# Autodesk Inventor assembly: RC Car Final Model
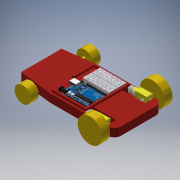
[picture p0: Inventor's stored thumbnail of the model, 180x180]
Saved by Autodesk Inventor 2019 (Build 230136000, 136)
## iProperties
Created: 2020-12-19
Part Number: RC Car Final Model
Document SubType Name: Assembly
Designer: wahid
Author: wahid
## Documents named in this file (9)
- C:\Users\wahid\Desktop\rc\Final Assembly\RC Car Final Model.iam
- C:\Users\wahid\Desktop\rc\Parts\Chassis\RC_Chassis.ipt
- C:\Users\wahid\Desktop\rc\Parts\Arduino\ardino.ipt
- C:\Users\wahid\Desktop\rc\Parts\Bread Board\Breadboard part\HalfBreadboard.ipt
- C:\Users\wahid\Desktop\rc\Parts\Motor\Original\Hobby_GearMotor.ipt
- C:\Users\wahid\Desktop\rc\Parts\Axle\Back Axle\Back Axle.ipt
- C:\Users\wahid\Desktop\rc\Parts\Wheel\Back Wheel\Back Wheel.ipt
- C:\Users\wahid\Desktop\rc\Parts\Axle\Front Axle\Front Axle.ipt
- C:\Users\wahid\Desktop\rc\Parts\Wheel\Front Wheel\Front Wheel.ipt
## Components (12 placed, 8 different names)
1. RC_Chassis:1 — Mate:3, Mate:4, Mate:5, Flush:1, Mate:6, Mate:7, Flush:2, Mate:8, Mate:12, Mate:13, Mate:14, Mate:15
2. HalfBreadboard:1 — Mate:3, Mate:4, Mate:12, Flush:4
3. Hobby_GearMotor:1 — Mate:5, Flush:1, Mate:6, Mate:9
4. Hobby_GearMotor:2 — Mate:7, Flush:2, Mate:8, Mate:10
5. Back Axle:1 — Mate:9, Insert:1
6. Back Axle:2 — Mate:10, Insert:2
7. Back Wheel:1 — Insert:1
8. Back Wheel:2 — Insert:2
9. Front Axle:1 — Mate:13, Insert:4, Insert:5
10. Front Wheel:2 — Insert:4
11. ardino:1 — Mate:14, Flush:4
12. Front Wheel:3 — Insert:5, Mate:15
## Relationships (19: Mate 12, Insert 4, Flush 3)
- Mate:3: RC_Chassis:1 ↔ HalfBreadboard:1
- Mate:4: RC_Chassis:1 ↔ HalfBreadboard:1
- Mate:5: RC_Chassis:1 ↔ Hobby_GearMotor:1
- Flush:1: RC_Chassis:1 ↔ Hobby_GearMotor:1
- Mate:6: RC_Chassis:1 ↔ Hobby_GearMotor:1
- Mate:7: RC_Chassis:1 ↔ Hobby_GearMotor:2
- Flush:2: RC_Chassis:1 ↔ Hobby_GearMotor:2
- Mate:8: RC_Chassis:1 ↔ Hobby_GearMotor:2
- Mate:9: Hobby_GearMotor:1 ↔ Back Axle:1
- Mate:10: Hobby_GearMotor:2 ↔ Back Axle:2
- Insert:1: Back Axle:1 ↔ Back Wheel:1
- Insert:2: Back Axle:2 ↔ Back Wheel:2
- Mate:12: RC_Chassis:1 ↔ HalfBreadboard:1
- Mate:13: RC_Chassis:1 ↔ Front Axle:1
- Insert:4: Front Axle:1 ↔ Front Wheel:2
- Mate:14: RC_Chassis:1 ↔ ardino:1
- Flush:4: HalfBreadboard:1 ↔ ardino:1
- Insert:5: Front Axle:1 ↔ Front Wheel:3
- Mate:15 (14.732 mm): RC_Chassis:1 ↔ Front Wheel:3
